# Autodesk Inventor assembly: Outer
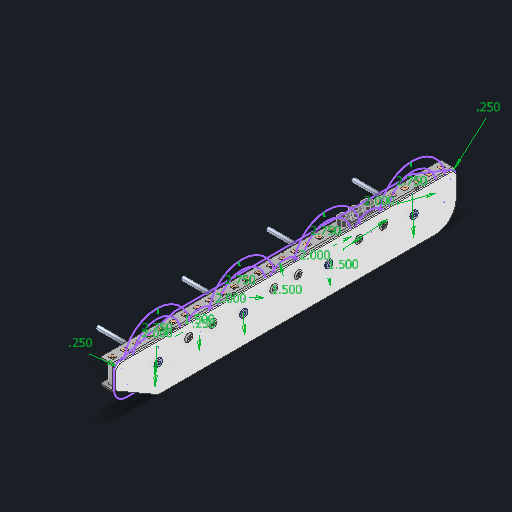
[picture p0: Inventor's stored thumbnail of the model, 512x512]
Saved by Autodesk Inventor 2025.1 (Build 291241000, 241)
## iProperties
Created: 2024-12-17
Part Number: Outer
Document SubType Name: Assembly
Designer: avere
Author: avere
## Documents named in this file (12)
- C:\Users\avere\VEX\High Stakes\CAD\V4\Chassis\Drivebay Left\Outer.iam
- C:\Users\avere\VEX\High Stakes\CAD\ROBOPROS-CAD-Inventor\Structure\C Channel\Aluminum 1x2x1\Alu C 1x2x1x28.ipt
- C:\Users\avere\VEX\High Stakes\CAD\V4\Chassis\Drivebay Left\Custom Parts\Skirt.ipt
- C:\Users\avere\VEX\High Stakes\CAD\ROBOPROS-CAD-Inventor\Structure\Hardware\Screw Steel - Star\SScrew Star Smooth 2.500.ipt
- C:\Users\avere\VEX\High Stakes\CAD\ROBOPROS-CAD-Inventor\Structure\Hardware\Nut Keps.ipt
- C:\Users\avere\VEX\High Stakes\CAD\ROBOPROS-CAD-Inventor\Structure\Hardware\Screw Nylon - Pan Head\NScrew Pan Head Threaded .500.ipt
- C:\Users\avere\VEX\High Stakes\CAD\ROBOPROS-CAD-Inventor\Structure\Hardware\Nut Nylon Thread-Forming.ipt
- C:\Users\avere\VEX\High Stakes\CAD\ROBOPROS-CAD-Inventor\Motion\Shaft LS\Bearing Flat Low Profile.ipt
- C:\Users\avere\VEX\High Stakes\CAD\ROBOPROS-CAD-Inventor\Structure\Nylon Standoff Rounded\Nylon Standoff .875.ipt
- C:\Users\avere\VEX\High Stakes\CAD\ROBOPROS-CAD-Inventor\Structure\Hardware\Screw Steel - Star.ipt
- C:\Users\avere\VEX\High Stakes\CAD\ROBOPROS-CAD-Inventor\Motion\Shaft LS\Bearing Flat.ipt
- C:\Users\avere\VEX\High Stakes\CAD\ROBOPROS-CAD-Inventor\Structure\1-Post Hex Nut Retainer With Nylon Hardware.iam
## Components (31 placed, 10 different names)
1. Alu C 1x2x1x28:1 — Flush:1, Flush:2, Flush:3, Insert:8, Mate:2, Insert:9, Insert:10, Mate:3, Insert:11, Insert:12, Mate:4, Insert:13, Mate:5, Insert:14, Insert:15, Insert:16
2. Skirt:1 — Insert:2, Insert:4, Insert:5, Insert:10, Mate:3
3. Nylon Standoff .875:1 — Insert:9
4. Bearing Flat:1 — Insert:12, Mate:4
5. 1-Post Hex Nut Retainer With Nylon Hardware:1 [sub-assembly] — Insert:13, Mate:5
6. Nut Keps:5 — Insert:14
7. Nut Keps:6 — Insert:15
8. Nut Nylon Thread-Forming:7 — Insert:16
9. Bearing Flat Low Profile:1 — Insert:6, Insert:7, Insert:8, Mate:2
10. Nut Nylon Thread-Forming:2 — Insert:7
11. Nut Nylon Thread-Forming:1 — Insert:6
12. NScrew Pan Head Threaded .500:2 — Insert:5
13. NScrew Pan Head Threaded .500:1 — Insert:4
14. Bearing Flat Low Profile:2
15. Nut Nylon Thread-Forming:3
16. Nut Nylon Thread-Forming:4
17. NScrew Pan Head Threaded .500:3
18. NScrew Pan Head Threaded .500:4
19. Bearing Flat Low Profile:3
20. Nut Nylon Thread-Forming:5
21. Nut Nylon Thread-Forming:6
22. NScrew Pan Head Threaded .500:5
23. NScrew Pan Head Threaded .500:6
24. Nut Keps:1 — Insert:11
25. SScrew Star Smooth 2.500:1 — Insert:2
26. Nut Keps:2
27. SScrew Star Smooth 2.500:2
28. Nut Keps:3
29. SScrew Star Smooth 2.500:3
30. Nut Keps:4
31. SScrew Star Smooth 2.500:4
## Component patterns: Bearings (3 elements), (4 elements, first: Nut Keps:1 + SScrew Star Smooth 2.500:1)
## Relationships (21: Insert 14, Mate 4, Flush 3)
- Flush:1 (-177.8 mm): Alu C 1x2x1x28:1
- Flush:2 (-12.7 mm): Alu C 1x2x1x28:1
- Flush:3 (-7.9375 mm): Alu C 1x2x1x28:1
- Insert:2: Skirt:1 ↔ SScrew Star Smooth 2.500:1
- Insert:4 (-1.5875 mm): Skirt:1 ↔ NScrew Pan Head Threaded .500:1
- Insert:5 (-1.5875 mm): Skirt:1 ↔ NScrew Pan Head Threaded .500:2
- Insert:6 (1.27 mm): Bearing Flat Low Profile:1 ↔ Nut Nylon Thread-Forming:1
- Insert:7 (1.27 mm): Bearing Flat Low Profile:1 ↔ Nut Nylon Thread-Forming:2
- Insert:8: Alu C 1x2x1x28:1 ↔ Bearing Flat Low Profile:1
- Mate:2: Alu C 1x2x1x28:1 ↔ Bearing Flat Low Profile:1
- Insert:9: Alu C 1x2x1x28:1 ↔ Nylon Standoff .875:1
- Insert:10: Alu C 1x2x1x28:1 ↔ Skirt:1
- Mate:3: Alu C 1x2x1x28:1 ↔ Skirt:1
- Insert:11: Alu C 1x2x1x28:1 ↔ Nut Keps:1
- Insert:12: Alu C 1x2x1x28:1 ↔ Bearing Flat:1
- Mate:4: Alu C 1x2x1x28:1 ↔ Bearing Flat:1
- Insert:13: Alu C 1x2x1x28:1 ↔ 1-Post Hex Nut Retainer With Nylon Hardware:1
- Mate:5: Alu C 1x2x1x28:1 ↔ 1-Post Hex Nut Retainer With Nylon Hardware:1
- Insert:14: Alu C 1x2x1x28:1 ↔ Nut Keps:5
- Insert:15: Alu C 1x2x1x28:1 ↔ Nut Keps:6
- Insert:16: Alu C 1x2x1x28:1 ↔ Nut Nylon Thread-Forming:7
